# Autodesk Inventor assembly: Assembly
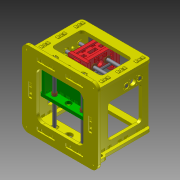
[picture p0: Inventor's stored thumbnail of the model, 180x180]
Saved by Autodesk Inventor 2012 SP1 (Build 160190100, 190)
## iProperties
Created: 2011-11-06
Part Number: Assembly
Document SubType Name: Assembly
Designer: Aaron
Author: Aaron
## Documents named in this file (4)
- C:\Users\Aaron\Documents\Projects\MTM-Snap-Metric\Assembly.iam
- C:\Users\Aaron\Documents\Projects\MTM-Snap-Metric\frame.iam
- C:\Users\Aaron\Documents\Projects\MTM-Snap-Metric\floor.iam
- C:\Users\Aaron\Documents\Projects\MTM-Snap-Metric\gantry.iam
## Components (3 placed, 3 different names)
1. frame:1 [sub-assembly] — Mate:1, Mate:2, Mate:3, Mate:4, Mate:5, Mate:6, Mate:7, Mate:8
2. floor:1 [sub-assembly] — Mate:1, Mate:2
3. gantry:1 [sub-assembly] — Mate:3, Mate:4, Mate:5, Mate:6, Mate:7, Mate:8
## Relationships (8: Mate 8)
- Mate:1: frame:1 ↔ floor:1
- Mate:2 (100 mm): frame:1 ↔ floor:1
- Mate:3: frame:1 ↔ gantry:1
- Mate:4: frame:1 ↔ gantry:1
- Mate:5: frame:1 ↔ gantry:1
- Mate:6: frame:1 ↔ gantry:1
- Mate:7: frame:1 ↔ gantry:1
- Mate:8: frame:1 ↔ gantry:1
